# Autodesk Inventor assembly: Cocei g. Janina constantina-T7
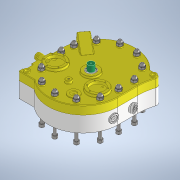
[picture p0: Inventor's stored thumbnail of the model, 180x180]
Saved by Autodesk Inventor 2022 (Build 260153000, 153)
## iProperties
Created: 2022-02-17
Part Number: Cocei g. Janina constantina-T7
Document SubType Name: Assembly
Designer: cteis
Author: cteis
## Documents named in this file (9)
- C:\Users\Janina\Desktop\CoceiJ\7 - Wankel\Cocei g. Janina constantina-T7.iam
- C:\Users\Janina\Desktop\CoceiJ\7 - Wankel\CapacSpate.ipt
- C:\Users\Janina\Desktop\CoceiJ\7 - Wankel\StatorWankel.ipt
- C:\Users\Janina\Desktop\CoceiJ\7 - Wankel\Arbore.ipt
- C:\Users\Janina\Desktop\CoceiJ\7 - Wankel\SansRotor.iam
- C:\Users\Janina\Desktop\CoceiJ\7 - Wankel\SansCapacFata.iam
- C:\Users\Janina\Desktop\CoceiJ\7 - Wankel\Ans Piulite Fixare.iam
- C:\Users\Janina\Desktop\CoceiJ\7 - Wankel\Ans Surub Fixare.iam
- D:\My Documents\Inventor\Content Center Files\R2022\en-US\ISO 6194 1  T 1\ISO 6194_1 - Type1 22 x 35 x 7.ipt
## Components (9 placed, 8 different names)
1. CapacSpate:1 — Mate:1, Mate:2, Angle:1, Mate:3, Mate:4, Mate:5, Mate:12
2. StatorWankel:1 — Mate:1, Mate:2, Angle:1, Unghi Animatie, Mate:10, Mate:11
3. Arbore:1 — Mate:3, Mate:4, Unghi Animatie, Mate:6, Mate:7, Rotation:1, Mate:9, Mate:13, Mate:15
4. SansRotor:1 [sub-assembly] — Mate:5, Mate:6, Mate:7, Rotation:1
5. SansCapacFata:1 [sub-assembly] — Mate:9, Mate:10, Mate:11, Mate:14
6. Ans Piulite Fixare:1 [sub-assembly]
7. Ans Surub Fixare:1 [sub-assembly]
8. ISO 6194/1 Type 1 Type1 22 x 35 x 7:1 — Mate:12, Mate:13
9. ISO 6194/1 Type 1 Type1 22 x 35 x 7:2 — Mate:14, Mate:15
## Relationships (19: Mate 14, Angle 2, Insert 2, RelateRotation 1)
- Mate:1: CapacSpate:1 ↔ StatorWankel:1
- Mate:2: CapacSpate:1 ↔ StatorWankel:1
- Angle:1 (0 deg): CapacSpate:1 ↔ StatorWankel:1
- Mate:3 (1 mm): CapacSpate:1 ↔ Arbore:1
- Mate:4: CapacSpate:1 ↔ Arbore:1
- Unghi Animatie [Angle] (1080 deg): StatorWankel:1 ↔ Arbore:1
- Mate:5: CapacSpate:1 ↔ SansRotor:1
- Mate:6: Arbore:1 ↔ SansRotor:1
- Mate:7: Arbore:1 ↔ SansRotor:1
- Rotation:1 [RelateRotation] (0.33 ul): Arbore:1 ↔ SansRotor:1
- Mate:9: Arbore:1 ↔ SansCapacFata:1
- Mate:10: StatorWankel:1 ↔ SansCapacFata:1
- Mate:11: StatorWankel:1 ↔ SansCapacFata:1
- [Insert]: SansCapacFata:1 ↔ Ans Surub Fixare:1
- [Insert]: CapacSpate:1 ↔ Ans Piulite Fixare:1
- Mate:12: CapacSpate:1 ↔ ISO 6194/1 Type 1 Type1 22 x 35 x 7:1
- Mate:13: Arbore:1 ↔ ISO 6194/1 Type 1 Type1 22 x 35 x 7:1
- Mate:14: SansCapacFata:1 ↔ ISO 6194/1 Type 1 Type1 22 x 35 x 7:2
- Mate:15: Arbore:1 ↔ ISO 6194/1 Type 1 Type1 22 x 35 x 7:2
